# Autodesk Inventor assembly: populated-keyboard_cherrymx
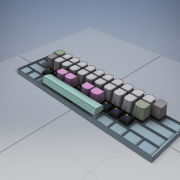
[picture p0: Inventor's stored thumbnail of the model, 180x180]
Saved by Autodesk Inventor 2016 (Build 200138000, 138)
## iProperties
Created: 2016-12-08
Part Number: populated-keyboard_cherrymx
Document SubType Name: Assembly
Designer: Cemra JC
Author: Cemra JC
## Documents named in this file (9)
- J:\The Files\The Software Files\Projects\stenotoppers\cherrymx\base-model\populated-keyboard_cherrymx.iam
- J:\The Files\The Software Files\Projects\stenotoppers\cherrymx\base-model\keyboard-mockup_cherrymx.iam
- J:\The Files\The Software Files\Projects\stenotoppers\cherrymx\base-model\standard-keycap_top-rows_base_cherrymx.ipt
- J:\The Files\The Software Files\Projects\stenotoppers\cherrymx\base-model\keyswitch_cherrymx.iam
- J:\The Files\The Software Files\Projects\stenotoppers\cherrymx\base-model\smaller-keycap_top-rows_base_cherrymx.ipt
- J:\The Files\The Software Files\Projects\stenotoppers\cherrymx\base-model\larger-keycap_top-rows_base_cherrymx.ipt
- J:\The Files\The Software Files\Projects\stenotoppers\cherrymx\base-model\spacebar-keycap_mockup_cherrymx.ipt
- J:\The Files\The Software Files\Projects\stenotoppers\cherrymx\base-model\thumb-keycap_thumb-row_base_cherrymx.ipt
- J:\The Files\The Software Files\Projects\stenotoppers\parameters.xlsx
## Components (30 placed, 7 different names)
1. keyboard-mockup_cherrymx:1 [sub-assembly] — Rigid:3, Rigid:4, Rigid:5, Rigid:6, Rigid:7, Rigid:8, Rigid:9, Rigid:11, Rigid:12
2. keyswitch_cherrymx:1 [sub-assembly] — Rigid:5, Rigid:10
3. smaller-keycap_top-rows_base_cherrymx:1 — Rigid:7
4. smaller-keycap_top-rows_base_cherrymx:2 — Rigid:6
5. larger-keycap_top-rows_base_cherrymx:1 — Rigid:8
6. larger-keycap_top-rows_base_cherrymx:2 — Rigid:9
7. spacebar-keycap_mockup_cherrymx:1 — Rigid:10
8. standard-keycap_top-rows_base_cherrymx:4 — Rigid:3
9. standard-keycap_top-rows_base_cherrymx:5
10. standard-keycap_top-rows_base_cherrymx:6
11. standard-keycap_top-rows_base_cherrymx:7
12. standard-keycap_top-rows_base_cherrymx:8
13. standard-keycap_top-rows_base_cherrymx:9
14. standard-keycap_top-rows_base_cherrymx:10
15. standard-keycap_top-rows_base_cherrymx:11
16. standard-keycap_top-rows_base_cherrymx:12
17. standard-keycap_top-rows_base_cherrymx:13
18. standard-keycap_top-rows_base_cherrymx:2 — Rigid:4
19. standard-keycap_top-rows_base_cherrymx:14
20. standard-keycap_top-rows_base_cherrymx:15
21. standard-keycap_top-rows_base_cherrymx:16
22. standard-keycap_top-rows_base_cherrymx:17
23. standard-keycap_top-rows_base_cherrymx:18
24. standard-keycap_top-rows_base_cherrymx:19
25. standard-keycap_top-rows_base_cherrymx:20
26. standard-keycap_top-rows_base_cherrymx:21
27. thumb-keycap_thumb-row_base_cherrymx:2 — Rigid:12
28. thumb-keycap_thumb-row_base_cherrymx:3
29. thumb-keycap_thumb-row_base_cherrymx:1 — Rigid:11
30. thumb-keycap_thumb-row_base_cherrymx:4
## Component patterns: (10 elements, first: standard-keycap_top-rows_base_cherrymx:4), (9 elements, first: standard-keycap_top-rows_base_cherrymx:2), (2 elements, first: thumb-keycap_thumb-row_base_cherrymx:2), (2 elements, first: thumb-keycap_thumb-row_base_cherrymx:1)
## Relationships (10: WeldJoint 10)
- Rigid:3 [WeldJoint]: keyboard-mockup_cherrymx:1 ↔ standard-keycap_top-rows_base_cherrymx:4
- Rigid:4 [WeldJoint]: keyboard-mockup_cherrymx:1 ↔ standard-keycap_top-rows_base_cherrymx:2
- Rigid:5 [WeldJoint]: keyboard-mockup_cherrymx:1 ↔ keyswitch_cherrymx:1
- Rigid:6 [WeldJoint]: keyboard-mockup_cherrymx:1 ↔ smaller-keycap_top-rows_base_cherrymx:2
- Rigid:7 [WeldJoint]: keyboard-mockup_cherrymx:1 ↔ smaller-keycap_top-rows_base_cherrymx:1
- Rigid:8 [WeldJoint]: keyboard-mockup_cherrymx:1 ↔ larger-keycap_top-rows_base_cherrymx:1
- Rigid:9 [WeldJoint]: keyboard-mockup_cherrymx:1 ↔ larger-keycap_top-rows_base_cherrymx:2
- Rigid:10 [WeldJoint]: keyswitch_cherrymx:1 ↔ spacebar-keycap_mockup_cherrymx:1
- Rigid:11 [WeldJoint]: keyboard-mockup_cherrymx:1 ↔ thumb-keycap_thumb-row_base_cherrymx:1
- Rigid:12 [WeldJoint]: keyboard-mockup_cherrymx:1 ↔ thumb-keycap_thumb-row_base_cherrymx:2
## Named parameters: k_width = 18.1 mm, k_height = 18 mm, k_height_t = 16 mm, k_taper1 = 1.5 mm, k_taper2 = 0.5 mm, k_staper = 1 mm, k_sradius = 4 mm, k_ltaper = 1.5 mm, k_lradius = 6 mm, k_radius = 6 mm, k_wthick = 1.5 mm, k_ribthick = 1.5 mm, k_ribheight = 5 mm, k_poleoff = 2.2625 mm, k_poledia = 5.54 mm, k_cmxw = 1.35 mm, k_cmxl = 4.4 mm, s_bwidth = 15.6 mm, s_poleh = 3.6 mm, s_polebw = 5.5 mm, s_polebl = 7 mm, b_pad = 1 mm, b_tab = 27.15 mm, b_caps = 31.675 mm, b_lshift = 40.725 mm, b_rshift = 49.775 mm, b_ctrl = 22.625 mm, b_space = 117.65 mm, b_width = 286.5 mm, b_height = 77.4 mm
